# Autodesk Inventor assembly: GripperV2
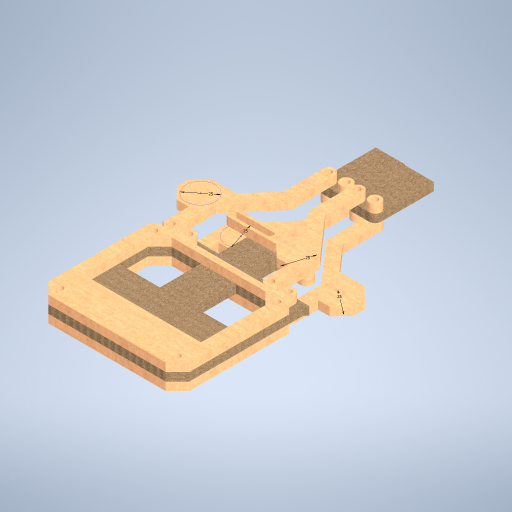
[picture p0: Inventor's stored thumbnail of the model, 512x512]
Saved by Autodesk Inventor 2023.1 (Build 271208000, 208)
## iProperties
Created: 2022-10-30
Part Number: GripperV2
Document SubType Name: Assembly
Designer: Daniel Peña
Author: Daniel Peña
## Documents named in this file (8)
- E:\Daniel DiscoA\Documents\UNAL\ProyectoRobotica\CAD\V2\GripperV2.iam
- E:\Daniel DiscoA\Documents\UNAL\ProyectoRobotica\CAD\V2\MarcoV2.ipt
- E:\Daniel DiscoA\Documents\UNAL\ProyectoRobotica\CAD\V2\PistonV2.ipt
- E:\Daniel DiscoA\Documents\UNAL\ProyectoRobotica\CAD\V2\BrazoTV2.ipt
- E:\Daniel DiscoA\Documents\UNAL\ProyectoRobotica\CAD\V2\BrazoV2.ipt
- E:\Daniel DiscoA\Documents\UNAL\ProyectoRobotica\CAD\V2\DedoV2.ipt
- E:\Daniel DiscoA\Documents\UNAL\ProyectoRobotica\CAD\V2\Tapa.ipt
- E:\Daniel DiscoA\Documents\UNAL\ProyectoRobotica\CAD\V2\Spacer.ipt
## Components (14 placed, 7 different names)
1. MarcoV2:1 — Rotational:1, Rotational:2, Rotational:3, Rotational:4, Piston, Flush:1, Rigid:1
2. PistonV2:1 — Piston
3. BrazoTV2:1 — Rotational:2, Rotational:6
4. BrazoTV2:2 — Rotational:1, Rotational:8
5. BrazoV2:1 — Rotational:4, Rotational:7
6. BrazoV2:2 — Rotational:3, Rotational:5
7. DedoV2:1 — Rotational:5, Rotational:8, Rigid:3, Rigid:4
8. DedoV2:2 — Rotational:6, Rotational:7, Rigid:2, Rigid:5
9. Tapa:1 — Flush:1
10. Tapa:2 — Rigid:1
11. Spacer:1 — Rigid:4
12. Spacer:2 — Rigid:3
13. Spacer:3 — Rigid:2
14. Spacer:4 — Rigid:5
## Relationships (15: RevoluteJoint 8, WeldJoint 5, TranslationJoint 1, Flush 1)
- Rotational:1 [RevoluteJoint]: MarcoV2:1 ↔ BrazoTV2:2
- Rotational:2 [RevoluteJoint]: MarcoV2:1 ↔ BrazoTV2:1
- Rotational:3 [RevoluteJoint]: MarcoV2:1 ↔ BrazoV2:2
- Rotational:4 [RevoluteJoint]: MarcoV2:1 ↔ BrazoV2:1
- Rotational:5 [RevoluteJoint]: BrazoV2:2 ↔ DedoV2:1
- Rotational:6 [RevoluteJoint]: BrazoTV2:1 ↔ DedoV2:2
- Rotational:7 [RevoluteJoint]: BrazoV2:1 ↔ DedoV2:2
- Rotational:8 [RevoluteJoint]: BrazoTV2:2 ↔ DedoV2:1
- Piston [TranslationJoint]: MarcoV2:1 ↔ PistonV2:1
- Flush:1: MarcoV2:1 ↔ Tapa:1
- Rigid:1 [WeldJoint]: MarcoV2:1 ↔ Tapa:2
- Rigid:2 [WeldJoint]: DedoV2:2 ↔ Spacer:3
- Rigid:3 [WeldJoint]: DedoV2:1 ↔ Spacer:2
- Rigid:4 [WeldJoint]: DedoV2:1 ↔ Spacer:1
- Rigid:5 [WeldJoint]: DedoV2:2 ↔ Spacer:4
